# Autodesk Inventor assembly: Chassis
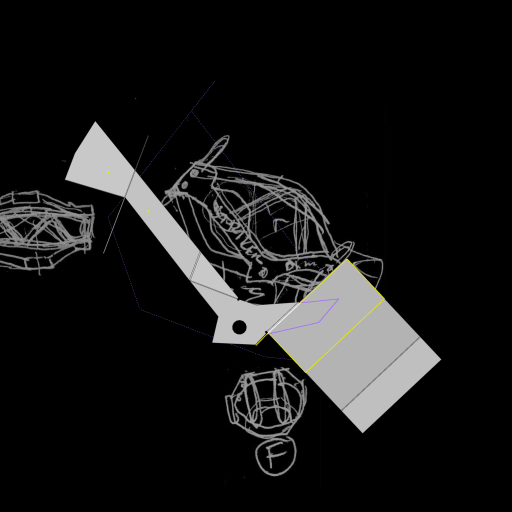
[picture p0: Inventor's stored thumbnail of the model, 512x512]
Saved by Autodesk Inventor 2023 (Build 270158000, 158)
## iProperties
Created: 2023-04-04
Part Number: Chassis
Document SubType Name: Assembly
Designer: valer
Author: valer
## Documents named in this file (3)
- C:\Users\valer\Desktop\str1ker\cad\Chassis.iam
- C:\Users\valer\Desktop\str1ker\cad\ChassisLeft.ipt
- C:\Users\valer\Desktop\str1ker\cad\ChassisRight.ipt
## Components (2 placed, 2 different names)
1. ChassisLeft:1 — Flush:3
2. ChassisRight:1 — Mate:1
## Relationships (3: Flush 2, Mate 1)
- Flush:1 (-248 mm)
- Flush:3: ChassisLeft:1
- Mate:1: ChassisRight:1
